# Autodesk Inventor assembly: tower1.3-01
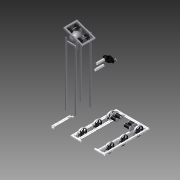
[picture p0: Inventor's stored thumbnail of the model, 180x180]
Saved by Autodesk Inventor 2011 SP1 (Build 150282100, 282)
## iProperties
Created: 2012-01-14
Part Number: tower1.3-01
Document SubType Name: Assembly
Designer: Christopher
Author: Christopher
## Documents named in this file (17)
- C:\Users\Christopher\Documents\Christopher\FIRST\Inventor files\2012\4 wheel kicker version 1\tower1.4.iam
- C:\Users\Christopher\Documents\Christopher\FIRST\Inventor files\2012\4 wheel kicker version 1\9 in .125 aluminum tube.ipt
- C:\Users\Christopher\Documents\Christopher\FIRST\Inventor files\2012\4 wheel kicker version 1\18 inch tube.ipt
- C:\Users\Christopher\Documents\Christopher\FIRST\Inventor files\2012\4 wheel kicker version 1\wheel.ipt
- C:\Users\Christopher\Documents\Christopher\FIRST\Inventor files\2012\4 wheel kicker version 1\axle1 .5inch.ipt
- C:\Users\Christopher\Documents\Christopher\FIRST\Inventor files\2012\tower first design\towerfrontdraft.ipt
- C:\Users\Christopher\Documents\Christopher\FIRST\Inventor files\2012\tower first design\towerbracebackwards.ipt
- C:\Users\Christopher\Documents\Christopher\FIRST\Inventor files\2012\tower first design\short thing.ipt
- C:\Users\Christopher\Documents\Christopher\FIRST\Inventor files\2012\tower first design\doorstop.ipt
- C:\Users\Christopher\Documents\Christopher\FIRST\Inventor files\2012\tower first design\towertallbackthing.ipt
- C:\Users\Christopher\Documents\Christopher\FIRST\Inventor files\2011\Kit of Parts\motors\Motors_FisherPrice_00968-9015.iam
- C:\Users\Christopher\Documents\Christopher\FIRST\Inventor files\2012\tower first design\pvc pipe 7inch.ipt
- C:\Users\Christopher\Documents\Christopher\FIRST\Inventor files\2011\Kit of Parts\Chassis\Chassis_CornerConnect_AndyMark_am-0212.ipt
- C:\Users\Christopher\Documents\Christopher\FIRST\Inventor files\2012\4 wheel kicker version 1\game ball.ipt
- C:\Users\Christopher\Documents\Christopher\FIRST\Inventor files\2012\robot base.iam
- C:\Users\Christopher\Documents\Christopher\FIRST\Inventor files\2011\Kit of Parts\Chassis\chassis 15 inch.ipt
- tower1-01.iam
## Components (28 placed, 15 different names)
1. 18 inch tube:2 — Insert:1, Insert:2, Mate:1, Flush:1, Flush:2, Flush:3, Mate:6, Flush:12, Insert:17
2. wheel:1 — Insert:3
3. wheel:2 — Insert:4
4. wheel:3 — Insert:9
5. wheel:4 — Insert:10
6. axle1 .5inch:1 — Insert:1, Insert:3, Insert:9
7. axle1 .5inch:2 — Insert:2, Insert:4, Insert:10
8. 9 in .125 aluminum tube:1 — Mate:1, Flush:1, Flush:2, Mate:17, Flush:27, Flush:28
9. 9 in .125 aluminum tube:2 — Flush:3, Mate:6, Flush:12
10. towerfrontdraft:1 — Mate:10, Flush:19, Flush:20
11. towerfrontdraft:2 — Mate:9, Flush:17, Flush:18, Mate:18
12. towerbracebackwards:1 — Mate:10, Flush:19, Flush:20, Mate:15, Flush:26, Mate:22, Mate:23, Mate:24, Mate:26, Flush:31, Flush:32
13. towerbracebackwards:2 — Mate:9, Flush:17, Flush:18, Mate:13, Flush:25, Mate:19, Mate:20, Mate:21, Mate:25, Flush:29, Flush:30
14. short thing:1 — Mate:13, Flush:25, Mate:18, Insert:17
15. short thing:2 — Mate:15, Flush:26
16. 18 inch tube:3 — Mate:17, Flush:27, Flush:28
17. doorstop:1 — Mate:19, Mate:20, Mate:21
18. doorstop:2 — Mate:22, Mate:23, Mate:24
19. towertallbackthing:1 — Mate:26, Flush:31, Flush:32
20. towertallbackthing:2 — Mate:25, Flush:29, Flush:30
21. Motors_FisherPrice_00968-9015:2 [sub-assembly] — Insert:16
22. pvc pipe 7inch:1 — Insert:16
23. pvc pipe 7inch:2
24. game ball:1
25. robot base:1 [sub-assembly]
26. chassis 15 inch:1 — Insert:18, Insert:19, Insert:20, Insert:21
27. Chassis_CornerConnect_AndyMark_am-0212:1 — Insert:20, Insert:21
28. Chassis_CornerConnect_AndyMark_am-0212:2 — Insert:18, Insert:19
## Relationships (44: Mate 16, Flush 16, Insert 12)
- Insert:1 (-12.7 mm): 18 inch tube:2 ↔ axle1 .5inch:1
- Insert:2 (-12.7 mm): 18 inch tube:2 ↔ axle1 .5inch:2
- Insert:3 (53.34 mm): wheel:1 ↔ axle1 .5inch:1
- Insert:4 (53.34 mm): wheel:2 ↔ axle1 .5inch:2
- Mate:1: 18 inch tube:2 ↔ 9 in .125 aluminum tube:1
- Flush:1: 18 inch tube:2 ↔ 9 in .125 aluminum tube:1
- Flush:2: 18 inch tube:2 ↔ 9 in .125 aluminum tube:1
- Insert:9 (193.04 mm): wheel:3 ↔ axle1 .5inch:1
- Insert:10 (193.04 mm): wheel:4 ↔ axle1 .5inch:2
- Flush:3: 18 inch tube:2 ↔ 9 in .125 aluminum tube:2
- Mate:6: 18 inch tube:2 ↔ 9 in .125 aluminum tube:2
- Flush:12: 18 inch tube:2 ↔ 9 in .125 aluminum tube:2
- Mate:9: towerfrontdraft:2 ↔ towerbracebackwards:2
- Flush:17: towerfrontdraft:2 ↔ towerbracebackwards:2
- Flush:18: towerfrontdraft:2 ↔ towerbracebackwards:2
- Mate:10: towerfrontdraft:1 ↔ towerbracebackwards:1
- Flush:19: towerfrontdraft:1 ↔ towerbracebackwards:1
- Flush:20: towerfrontdraft:1 ↔ towerbracebackwards:1
- Mate:13: towerbracebackwards:2 ↔ short thing:1
- Flush:25: towerbracebackwards:2 ↔ short thing:1
- Mate:15: towerbracebackwards:1 ↔ short thing:2
- Flush:26: towerbracebackwards:1 ↔ short thing:2
- Mate:17: 9 in .125 aluminum tube:1 ↔ 18 inch tube:3
- Flush:27: 9 in .125 aluminum tube:1 ↔ 18 inch tube:3
- Flush:28: 9 in .125 aluminum tube:1 ↔ 18 inch tube:3
- Mate:18 (-50.8 mm): towerfrontdraft:2 ↔ short thing:1
- Mate:19: towerbracebackwards:2 ↔ doorstop:1
- Mate:20 (-12.7 mm): towerbracebackwards:2 ↔ doorstop:1
- Mate:21 (-12.7 mm): towerbracebackwards:2 ↔ doorstop:1
- Mate:22: towerbracebackwards:1 ↔ doorstop:2
- Mate:23 (-12.7 mm): towerbracebackwards:1 ↔ doorstop:2
- Mate:24 (-12.7 mm): towerbracebackwards:1 ↔ doorstop:2
- Mate:25: towerbracebackwards:2 ↔ towertallbackthing:2
- Flush:29: towerbracebackwards:2 ↔ towertallbackthing:2
- Flush:30 (76.2 mm): towerbracebackwards:2 ↔ towertallbackthing:2
- Mate:26: towerbracebackwards:1 ↔ towertallbackthing:1
- Flush:31 (76.2 mm): towerbracebackwards:1 ↔ towertallbackthing:1
- Flush:32: towerbracebackwards:1 ↔ towertallbackthing:1
- Insert:16: Motors_FisherPrice_00968-9015:2 ↔ pvc pipe 7inch:1
- Insert:17: 18 inch tube:2 ↔ short thing:1
- Insert:18: chassis 15 inch:1 ↔ Chassis_CornerConnect_AndyMark_am-0212:2
- Insert:19: chassis 15 inch:1 ↔ Chassis_CornerConnect_AndyMark_am-0212:2
- Insert:20: chassis 15 inch:1 ↔ Chassis_CornerConnect_AndyMark_am-0212:1
- Insert:21: chassis 15 inch:1 ↔ Chassis_CornerConnect_AndyMark_am-0212:1
